# Autodesk Inventor assembly: Наливатор
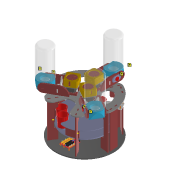
[picture p0: Inventor's stored thumbnail of the model, 180x180]
Saved by Autodesk Inventor 2022 (Build 260153000, 153)
## iProperties
Created: 2025-01-23
Part Number: Наливатор
Document SubType Name: Assembly
Designer: Ivan
Mass: 39441.3 g
Surface Area: 61367.1 cm^2
Volume: 38080.5 cm^3
Density: 1.03574 g/cm^3
Author: Ivan
Title: Наливатор
## Documents named in this file (7)
- E:\Предпроф 2025\Shoter_1_ZIP\Shoter_1.iam
- E:\Предпроф 2025\Shoter_1_ZIP\Рама.iam
- E:\Предпроф 2025\Shoter_1_ZIP\Узел емкости.iam
- E:\Предпроф 2025\Shoter_1_ZIP\Корпус_В2_Основание.ipt
- E:\Предпроф 2025\Shoter_1_ZIP\Nema17.iam
- E:\Предпроф 2025\Shoter_1_ZIP\Модуль перемещения.iam
- E:\Предпроф 2025\Shoter_1_ZIP\Кронштейн.iam
## Components (10 placed, 6 different names)
1. Рама:1 [sub-assembly] — Совмещение:1, Совмещение:2, Заподлицо:1, Совмещение:21, Совмещение:22
2. Узел емкости:1 [sub-assembly] — Совмещение:5, Совмещение:8, Совмещение:10
3. Узел емкости:2 [sub-assembly] — Совмещение:4, Совмещение:7, Совмещение:9
4. Узел емкости:3 [sub-assembly] — Совмещение:3, Совмещение:6, Совмещение:11
5. Корпус_В2_Основание:1 — Совмещение:1, Совмещение:2, Заподлицо:1, Совмещение:3, Совмещение:4, Совмещение:5, Совмещение:6, Совмещение:7, Совмещение:8, Совмещение:9, Совмещение:10, Совмещение:11, Совмещение:12, Совмещение:13, Совмещение:14, Совмещение:15, Совмещение:16, Совмещение:17, Совмещение:18, Совмещение:19, Совмещение:20, Совмещение:23, Совмещение:24, Совмещение:25
6. Насос:1 [sub-assembly] — Совмещение:12, Совмещение:19, Совмещение:20
7. Насос:2 [sub-assembly] — Совмещение:13, Совмещение:17, Совмещение:18
8. Насос:3 [sub-assembly] — Совмещение:14, Совмещение:15, Совмещение:16
9. Модуль перемещения:1 [sub-assembly] — Совмещение:21, Совмещение:22
10. Кронштейн:1 [sub-assembly] — Совмещение:23, Совмещение:24, Совмещение:25
## Relationships (26: Mate 25, Flush 1)
- Совмещение:1 [Mate]: Рама:1 ↔ Корпус_В2_Основание:1
- Совмещение:2 [Mate]: Рама:1 ↔ Корпус_В2_Основание:1
- Заподлицо:1 [Flush]: Рама:1 ↔ Корпус_В2_Основание:1
- Совмещение:3 [Mate]: Узел емкости:3 ↔ Корпус_В2_Основание:1
- Совмещение:4 [Mate]: Узел емкости:2 ↔ Корпус_В2_Основание:1
- Совмещение:5 [Mate]: Узел емкости:1 ↔ Корпус_В2_Основание:1
- Совмещение:6 [Mate]: Узел емкости:3 ↔ Корпус_В2_Основание:1
- Совмещение:7 [Mate]: Узел емкости:2 ↔ Корпус_В2_Основание:1
- Совмещение:8 [Mate]: Узел емкости:1 ↔ Корпус_В2_Основание:1
- Совмещение:9 [Mate]: Узел емкости:2 ↔ Корпус_В2_Основание:1
- Совмещение:10 [Mate]: Узел емкости:1 ↔ Корпус_В2_Основание:1
- Совмещение:11 [Mate]: Узел емкости:3 ↔ Корпус_В2_Основание:1
- Совмещение:12 [Mate]: Корпус_В2_Основание:1 ↔ Насос:1
- Совмещение:13 [Mate]: Корпус_В2_Основание:1 ↔ Насос:2
- Совмещение:14 [Mate]: Корпус_В2_Основание:1 ↔ Насос:3
- Совмещение:15 [Mate]: Корпус_В2_Основание:1 ↔ Насос:3
- Совмещение:16 [Mate]: Корпус_В2_Основание:1 ↔ Насос:3
- Совмещение:17 [Mate]: Корпус_В2_Основание:1 ↔ Насос:2
- Совмещение:18 [Mate]: Корпус_В2_Основание:1 ↔ Насос:2
- Совмещение:19 [Mate]: Корпус_В2_Основание:1 ↔ Насос:1
- Совмещение:20 [Mate]: Корпус_В2_Основание:1 ↔ Насос:1
- Совмещение:21 [Mate]: Рама:1 ↔ Модуль перемещения:1
- Совмещение:22 [Mate]: Рама:1 ↔ Модуль перемещения:1
- Совмещение:23 [Mate]: Корпус_В2_Основание:1 ↔ Кронштейн:1
- Совмещение:24 [Mate]: Корпус_В2_Основание:1 ↔ Кронштейн:1
- Совмещение:25 [Mate]: Корпус_В2_Основание:1 ↔ Кронштейн:1
